# Autodesk Inventor assembly: Sestava merilnika
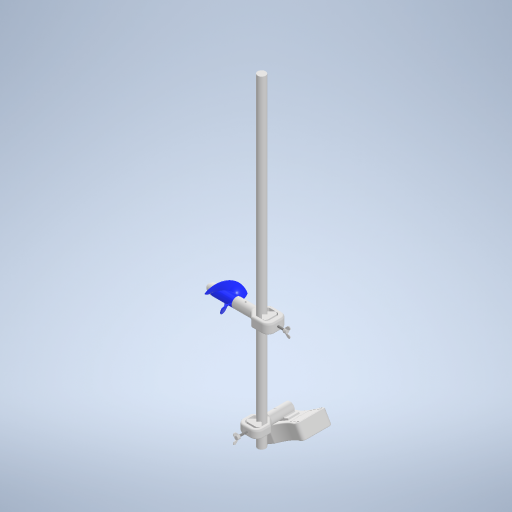
[picture p0: Inventor's stored thumbnail of the model, 512x512]
Saved by Autodesk Inventor 2023 (Build 270158000, 158)
## iProperties
Created: 2023-04-03
Part Number: Sestava merilnika
Document SubType Name: Assembly
Designer: Tone
Author: Tone
## Documents named in this file (14)
- E:\Projekti\Izdelki\FS\H hope\Sestava merilnika.iam
- E:\Projekti\Izdelki\FS\H hope\Rotor.ipt
- E:\Projekti\Izdelki\FS\H hope\Ležaj 608-2RSL.ipt
- E:\Projekti\Izdelki\FS\H hope\Držalo.ipt
- E:\Projekti\Izdelki\FS\H hope\Drsnik.ipt
- E:\Projekti\Izdelki\FS\H hope\Matica M6 x 1.ipt
- E:\Projekti\Izdelki\FS\H hope\Krilni vijak M6 x 40.ipt
- E:\Projekti\Izdelki\FS\H hope\Kapa.ipt
- E:\Projekti\Izdelki\FS\H hope\Drog.ipt
- E:\Projekti\Izdelki\FS\H hope\Sestava škatle.iam
- E:\Projekti\Izdelki\FS\H hope\Sestava držala.iam
- E:\Projekti\Izdelki\FS\H hope\Compress Spring11.ipt
- E:\Projekti\Izdelki\FS\H hope\Inbus M8 x 40.ipt
- E:\Projekti\Izdelki\FS\H hope\Podložka široka 8.ipt
## Components (15 placed, 13 different names)
1. Rotor:1 — Mate:1, Mate:2, Mate:3, Mate:4, Mate:6, Angle:1, Mate:12, Mate:13
2. Ležaj 608-2RSL:1 — Mate:1, Mate:2, Mate:5
3. Ležaj 608-2RSL:2 — Mate:3, Mate:4
4. Držalo:1 — Mate:5, Mate:6, Flush:1, Angle:1, Mate:7, Mate:8, Mate:9, Angle:2, Mate:11, Tangent:1, Tangent:2, Angle:3
5. Drsnik:1 — Flush:1, Mate:7, Mate:10, Tangent:3
6. Matica M6 x 1:1 — Mate:8, Mate:9, Angle:2
7. Krilni vijak M6 x 40:1 — Mate:10, Mate:11
8. Kapa:1 — Mate:12, Mate:13
9. Drog:1 — Tangent:1, Tangent:2, Tangent:3, Tangent:4, Tangent:5, Flush:4
10. Sestava škatle:1 [sub-assembly] — Mate:14, Flush:2, Flush:3
11. Sestava držala:1 [sub-assembly] — Tangent:4, Tangent:5, Angle:3, Mate:14, Flush:2, Flush:3, Flush:4, Mate:15, Mate:16, Mate:17, Mate:18, Mate:22
12. Krilni vijak M6 x 40:2 — Mate:15, Mate:16
13. Compress Spring1:1 — Mate:17, Mate:18, Mate:21
14. Inbus M8 x 40:1 — Mate:19, Mate:20, Mate:22
15. Podložka široka 8:1 — Mate:19, Mate:20, Mate:21
## Relationships (34: Mate 22, Tangent 5, Flush 4, Angle 3)
- Mate:1: Rotor:1 ↔ Ležaj 608-2RSL:1
- Mate:2: Rotor:1 ↔ Ležaj 608-2RSL:1
- Mate:3: Rotor:1 ↔ Ležaj 608-2RSL:2
- Mate:4: Rotor:1 ↔ Ležaj 608-2RSL:2
- Mate:5: Ležaj 608-2RSL:1 ↔ Držalo:1
- Mate:6: Rotor:1 ↔ Držalo:1
- Flush:1: Držalo:1 ↔ Drsnik:1
- Angle:1 (0 deg): Rotor:1 ↔ Držalo:1
- Mate:7: Držalo:1 ↔ Drsnik:1
- Mate:8: Držalo:1 ↔ Matica M6 x 1:1
- Mate:9: Držalo:1 ↔ Matica M6 x 1:1
- Angle:2 (0 deg): Držalo:1 ↔ Matica M6 x 1:1
- Mate:10: Drsnik:1 ↔ Krilni vijak M6 x 40:1
- Mate:11: Držalo:1 ↔ Krilni vijak M6 x 40:1
- Mate:12: Rotor:1 ↔ Kapa:1
- Mate:13: Rotor:1 ↔ Kapa:1
- Tangent:1: Držalo:1 ↔ Drog:1
- Tangent:2: Držalo:1 ↔ Drog:1
- Tangent:3: Drsnik:1 ↔ Drog:1
- Tangent:4: Drog:1 ↔ Sestava držala:1
- Tangent:5: Drog:1 ↔ Sestava držala:1
- Angle:3 (0 deg): Držalo:1 ↔ Sestava držala:1
- Mate:14: Sestava škatle:1 ↔ Sestava držala:1
- Flush:2 (-60 mm): Sestava škatle:1 ↔ Sestava držala:1
- Flush:3 (-30 mm): Sestava škatle:1 ↔ Sestava držala:1
- Flush:4 (-50 mm): Drog:1 ↔ Sestava držala:1
- Mate:15: Sestava držala:1 ↔ Krilni vijak M6 x 40:2
- Mate:16: Sestava držala:1 ↔ Krilni vijak M6 x 40:2
- Mate:17: Sestava držala:1 ↔ Compress Spring1:1
- Mate:18: Sestava držala:1 ↔ Compress Spring1:1
- Mate:19: Inbus M8 x 40:1 ↔ Podložka široka 8:1
- Mate:20: Inbus M8 x 40:1 ↔ Podložka široka 8:1
- Mate:21: Compress Spring1:1 ↔ Podložka široka 8:1
- Mate:22: Sestava držala:1 ↔ Inbus M8 x 40:1
